# Autodesk Inventor assembly: Computer equipment
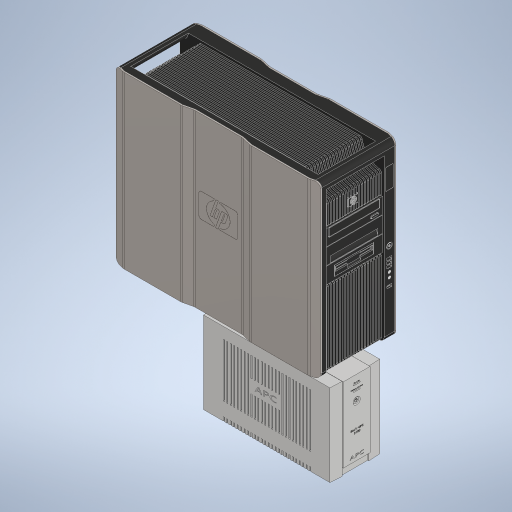
[picture p0: Inventor's stored thumbnail of the model, 512x512]
Saved by Autodesk Inventor 2024 (Build 280153000, 153)
## iProperties
Created: 2021-12-30
Part Number: Computer equipment
Document SubType Name: Assembly
Designer: sauliusd
Author: sauliusd
## Documents named in this file (3)
- C:\W4INV 2024 Design\PROJECTS\Samples\Macro DEMO\7 Computer Box\Computer equipment.iam
- C:\W4INV 2024 Design\PROJECTS\Samples\Macro DEMO\7 Computer Box\Z800\HP z800.iam
- C:\W4INV 2024 Design\PROJECTS\Samples\Macro DEMO\7 Computer Box\UPS\apc_bx1400u-gr.ipt
## Components (2 placed, 2 different names)
1. HP z800:1 [sub-assembly] — Mate:1, Flush:1, Flush:2, Mate:3
2. apc_bx1400u-gr:1 — Mate:2, Flush:2
## Relationships (5: Mate 3, Flush 2)
- Mate:1 (250 mm): HP z800:1
- Flush:1: HP z800:1
- Mate:2: apc_bx1400u-gr:1
- Flush:2: HP z800:1 ↔ apc_bx1400u-gr:1
- Mate:3: HP z800:1
